# Autodesk Inventor assembly: MAN_ASSEMBLY
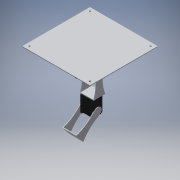
[picture p0: Inventor's stored thumbnail of the model, 180x180]
Saved by Autodesk Inventor 2019 (Build 230136000, 136)
## iProperties
Created: 2021-03-06
Part Number: MAN_ASSEMBLY
Document SubType Name: Assembly
Designer: DOMEK
Author: DOMEK
## Documents named in this file (5)
- D:\Manipulator\MAN_ASSEMBLY.iam
- D:\Manipulator\DYNAMIXEL_RX-18.ipt
- D:\Manipulator\MAN_BASIS_PLATE.ipt
- D:\Manipulator\MAN_BASIS_PRIMARY_STRUCTURE.ipt
- D:\Manipulator\MAN_BASIS_SECONDARY_STRUCTURE.ipt
## Components (7 placed, 4 different names)
1. DYNAMIXEL_RX-18:1 — Mate:1, Mate:2, Mate:15
2. MAN_BASIS_PLATE:1 — Mate:1, Mate:2
3. MAN_BASIS_SECONDARY_STRUCTURE:1 — Mate:15, Mate:16
4. DYNAMIXEL_RX-18:9 — Mate:16, Mate:17
5. MAN_BASIS_PRIMARY_STRUCTURE:1 — Mate:17, Mate:18, Flush:1, Flush:2
6. DYNAMIXEL_RX-18:10 — Mate:18, Flush:1, Flush:2, Mate:19
7. MAN_BASIS_PRIMARY_STRUCTURE:2 — Mate:19
## Relationships (9: Mate 7, Flush 2)
- Mate:1: DYNAMIXEL_RX-18:1 ↔ MAN_BASIS_PLATE:1
- Mate:2 (-115 mm): DYNAMIXEL_RX-18:1 ↔ MAN_BASIS_PLATE:1
- Mate:15: DYNAMIXEL_RX-18:1 ↔ MAN_BASIS_SECONDARY_STRUCTURE:1
- Mate:16: MAN_BASIS_SECONDARY_STRUCTURE:1 ↔ DYNAMIXEL_RX-18:9
- Mate:17: DYNAMIXEL_RX-18:9 ↔ MAN_BASIS_PRIMARY_STRUCTURE:1
- Mate:18: MAN_BASIS_PRIMARY_STRUCTURE:1 ↔ DYNAMIXEL_RX-18:10
- Flush:1: MAN_BASIS_PRIMARY_STRUCTURE:1 ↔ DYNAMIXEL_RX-18:10
- Flush:2: MAN_BASIS_PRIMARY_STRUCTURE:1 ↔ DYNAMIXEL_RX-18:10
- Mate:19: DYNAMIXEL_RX-18:10 ↔ MAN_BASIS_PRIMARY_STRUCTURE:2
